# Autodesk Inventor assembly: Assembly_Matchboxscope_injectionmolded_Anglerfish
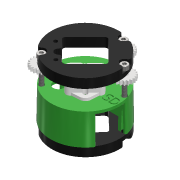
[picture p0: Inventor's stored thumbnail of the model, 180x180]
Saved by Autodesk Inventor 2022 (Build 260153000, 153)
## iProperties
Created: 2023-04-12
Part Number: Assembly_Matchboxscope_injectionmolded_Anglerfish
Document SubType Name: Assembly
Designer: diederichbenedict
Author: diederichbenedict
## Documents named in this file (11)
- C:\Users\diederichbenedict\Dropbox\Dokumente\Promotion\PROJECTS\Matchboxscope\INVENTOR\RELEASE\InjectionMolded\Assembly_Matchboxscope_injectionmolded_Anglerfish.iam
- C:\Users\diederichbenedict\Dropbox\Dokumente\Promotion\PROJECTS\Matchboxscope\INVENTOR\RELEASE\InjectionMolded\IM_Matchboxscope_base.ipt
- C:\Users\diederichbenedict\Dropbox\Dokumente\Promotion\PROJECTS\Matchboxscope\INVENTOR\RELEASE\InjectionMolded\IM_Matchboxscope_plate.ipt
- C:\Users\diederichbenedict\Dropbox\Dokumente\Promotion\PROJECTS\Matchboxscope\INVENTOR\RELEASE\InjectionMolded\IM_Periscope.ipt
- C:\Users\diederichbenedict\Dropbox\Dokumente\Promotion\PROJECTS\Matchboxscope\INVENTOR\RELEASE\InjectionMolded\Anglerfish_Cameraspacer.ipt
- C:\Users\diederichbenedict\Dropbox\Dokumente\Promotion\PROJECTS\Matchboxscope\INVENTOR\RELEASE\InjectionMolded\00_CCTV_M12_VCM_large.ipt
- C:\Users\diederichbenedict\Dropbox\Dokumente\Promotion\PROJECTS\Matchboxscope\INVENTOR\RELEASE\InjectionMolded\IM_Lensholder_M12.ipt
- C:\Users\diederichbenedict\Dropbox\Dokumente\Promotion\PROJECTS\Matchboxscope\INVENTOR\RELEASE\InjectionMolded\Matchboxscope_M12_Lensadapter_v0.ipt
- C:\Users\diederichbenedict\Dropbox\Dokumente\Promotion\PROJECTS\Matchboxscope\INVENTOR\RELEASE\InjectionMolded\00_Turningscrew.ipt
- C:\Users\diederichbenedict\Documents\Inventor\Content Center Files\R2022\de-DE\DIN 912\DIN 912 - M3 x 0.5 x 25 x 18.ipt
- C:\Users\diederichbenedict\Documents\Inventor\Content Center Files\R2022\de-DE\DIN 912\DIN 912 - M3 x 0.5 x 10 x 8.75.ipt
## Components (15 placed, 10 different names)
1. IM_Matchboxscope_base:1 — Einfügen:3, Passend:3, Einfügen:16, Einfügen:17
2. IM_Matchboxscope_plate:1 — Einfügen:10
3. IM_Periscope:1
4. Anglerfish_Cameraspacer:1
5. 00_CCTV_M12_VCM_large:1 — Einfügen:15
6. Matchboxscope_M12_Lensadapter_v0:1 — Einfügen:15, Einfügen:17
7. 00_Turningscrew:1 — Einfügen:11
8. IM_Matchboxscope_plate:2 — Einfügen:3, Passend:3, Einfügen:5, Einfügen:6, Einfügen:7, Einfügen:11, Einfügen:12, Einfügen:13
9. DIN 912 - ersetzt durch DIN EN ISO 4762 M3 x 25:1 — Einfügen:5
10. DIN 912 - ersetzt durch DIN EN ISO 4762 M3 x 25:2 — Einfügen:6
11. DIN 912 - ersetzt durch DIN EN ISO 4762 M3 x 25:3 — Einfügen:7
12. DIN 912 - ersetzt durch DIN EN ISO 4762 M3 x 10:1 — Einfügen:10
13. 00_Turningscrew:2 — Einfügen:13
14. 00_Turningscrew:3 — Einfügen:12
15. IM_Lensholder_M12:1 — Einfügen:16
## Relationships (14: Insert 13, Mate 1)
- [Insert]: IM_Matchboxscope_base:1 ↔ IM_Matchboxscope_plate:1
- [Insert]: IM_Matchboxscope_base:1 ↔ IM_Matchboxscope_plate:1
- Einfügen:3 [Insert] (15 mm): IM_Matchboxscope_base:1 ↔ IM_Matchboxscope_plate:2
- Passend:3 [Mate]: IM_Matchboxscope_base:1 ↔ IM_Matchboxscope_plate:2
- Einfügen:5 [Insert]: IM_Matchboxscope_plate:2 ↔ DIN 912 - ersetzt durch DIN EN ISO 4762 M3 x 25:1
- Einfügen:6 [Insert]: IM_Matchboxscope_plate:2 ↔ DIN 912 - ersetzt durch DIN EN ISO 4762 M3 x 25:2
- Einfügen:7 [Insert]: IM_Matchboxscope_plate:2 ↔ DIN 912 - ersetzt durch DIN EN ISO 4762 M3 x 25:3
- Einfügen:10 [Insert] (-4 mm): IM_Matchboxscope_plate:1 ↔ DIN 912 - ersetzt durch DIN EN ISO 4762 M3 x 10:1
- Einfügen:11 [Insert]: 00_Turningscrew:1 ↔ IM_Matchboxscope_plate:2
- Einfügen:12 [Insert]: IM_Matchboxscope_plate:2 ↔ 00_Turningscrew:3
- Einfügen:13 [Insert]: IM_Matchboxscope_plate:2 ↔ 00_Turningscrew:2
- Einfügen:15 [Insert] (2 mm): 00_CCTV_M12_VCM_large:1 ↔ Matchboxscope_M12_Lensadapter_v0:1
- Einfügen:16 [Insert]: IM_Matchboxscope_base:1 ↔ IM_Lensholder_M12:1
- Einfügen:17 [Insert]: IM_Matchboxscope_base:1 ↔ Matchboxscope_M12_Lensadapter_v0:1
